# Autodesk Inventor assembly: BBM Staging Plate Assembly
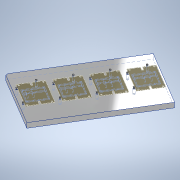
[picture p0: Inventor's stored thumbnail of the model, 180x180]
Saved by Autodesk Inventor 2022 (Build 260153000, 153)
## iProperties
Created: 2021-01-11
Part Number: BBM Staging Plate Assembly
Document SubType Name: Assembly
Designer: caleb
Author: caleb
## Documents named in this file (4)
- C:\Users\Caleb\Desktop\nebraska-silicon-lab\Hardware\ETL\Module Assembly\Baseplate Staging Plate - V1\Baseplate Staging Plate Assembly - V1.iam
- C:\Users\Caleb\Desktop\nebraska-silicon-lab\Hardware\ETL\Module Assembly\Baseplate Staging Plate - V1\Baseplate Staging Plate - V1.ipt
- C:\Users\Caleb\Desktop\nebraska-silicon-lab\Hardware\ETL\modules\etl standard baseplate with cutouts.ipt
- C:\Users\Caleb\Desktop\nebraska-silicon-lab\Hardware\ETL\Module Assembly\Baseplate Staging Plate - V1\98381A304_Dowel Pin.ipt
## Components (17 placed, 3 different names)
1. Baseplate Staging Plate - V1:1 — Mate:1, Mate:2, Mate:3, Mate:4, Insert:1, Insert:2, Insert:3, Insert:4, Insert:5, Insert:6, Insert:7, Insert:8, Insert:9, Insert:10, Insert:11, Insert:12
2. etl standard baseplate with cutouts:1 — Mate:1, Tangent:1, Tangent:2, Tangent:3
3. etl standard baseplate with cutouts:2 — Mate:2, Tangent:4, Tangent:5, Tangent:6
4. etl standard baseplate with cutouts:3 — Mate:3, Tangent:7, Tangent:8, Tangent:9
5. etl standard baseplate with cutouts:4 — Mate:4, Tangent:10, Tangent:11, Tangent:12
6. 98381A304_Dowel Pin:1 — Insert:3, Tangent:2
7. 98381A304_Dowel Pin:2 — Insert:1, Tangent:3
8. 98381A304_Dowel Pin:3 — Insert:2, Tangent:1
9. 98381A304_Dowel Pin:4 — Insert:4, Tangent:4
10. 98381A304_Dowel Pin:5 — Insert:5, Tangent:6
11. 98381A304_Dowel Pin:6 — Insert:6, Tangent:5
12. 98381A304_Dowel Pin:7 — Insert:7, Tangent:7
13. 98381A304_Dowel Pin:8 — Insert:8, Tangent:9
14. 98381A304_Dowel Pin:9 — Insert:9, Tangent:8
15. 98381A304_Dowel Pin:10 — Insert:10, Tangent:10
16. 98381A304_Dowel Pin:11 — Insert:11, Tangent:12
17. 98381A304_Dowel Pin:12 — Insert:12, Tangent:11
## Relationships (28: Insert 12, Tangent 12, Mate 4)
- Mate:1: Baseplate Staging Plate - V1:1 ↔ etl standard baseplate with cutouts:1
- Mate:2: Baseplate Staging Plate - V1:1 ↔ etl standard baseplate with cutouts:2
- Mate:3: Baseplate Staging Plate - V1:1 ↔ etl standard baseplate with cutouts:3
- Mate:4: Baseplate Staging Plate - V1:1 ↔ etl standard baseplate with cutouts:4
- Insert:1: Baseplate Staging Plate - V1:1 ↔ 98381A304_Dowel Pin:2
- Insert:2: Baseplate Staging Plate - V1:1 ↔ 98381A304_Dowel Pin:3
- Insert:3: Baseplate Staging Plate - V1:1 ↔ 98381A304_Dowel Pin:1
- Insert:4: Baseplate Staging Plate - V1:1 ↔ 98381A304_Dowel Pin:4
- Insert:5: Baseplate Staging Plate - V1:1 ↔ 98381A304_Dowel Pin:5
- Insert:6: Baseplate Staging Plate - V1:1 ↔ 98381A304_Dowel Pin:6
- Insert:7: Baseplate Staging Plate - V1:1 ↔ 98381A304_Dowel Pin:7
- Insert:8: Baseplate Staging Plate - V1:1 ↔ 98381A304_Dowel Pin:8
- Insert:9: Baseplate Staging Plate - V1:1 ↔ 98381A304_Dowel Pin:9
- Insert:10: Baseplate Staging Plate - V1:1 ↔ 98381A304_Dowel Pin:10
- Insert:11: Baseplate Staging Plate - V1:1 ↔ 98381A304_Dowel Pin:11
- Insert:12: Baseplate Staging Plate - V1:1 ↔ 98381A304_Dowel Pin:12
- Tangent:1: etl standard baseplate with cutouts:1 ↔ 98381A304_Dowel Pin:3
- Tangent:2: etl standard baseplate with cutouts:1 ↔ 98381A304_Dowel Pin:1
- Tangent:3: etl standard baseplate with cutouts:1 ↔ 98381A304_Dowel Pin:2
- Tangent:4: etl standard baseplate with cutouts:2 ↔ 98381A304_Dowel Pin:4
- Tangent:5: etl standard baseplate with cutouts:2 ↔ 98381A304_Dowel Pin:6
- Tangent:6: etl standard baseplate with cutouts:2 ↔ 98381A304_Dowel Pin:5
- Tangent:7: etl standard baseplate with cutouts:3 ↔ 98381A304_Dowel Pin:7
- Tangent:8: etl standard baseplate with cutouts:3 ↔ 98381A304_Dowel Pin:9
- Tangent:9: etl standard baseplate with cutouts:3 ↔ 98381A304_Dowel Pin:8
- Tangent:10: etl standard baseplate with cutouts:4 ↔ 98381A304_Dowel Pin:10
- Tangent:11: etl standard baseplate with cutouts:4 ↔ 98381A304_Dowel Pin:12
- Tangent:12: etl standard baseplate with cutouts:4 ↔ 98381A304_Dowel Pin:11
